# Autodesk Inventor assembly: Montagem
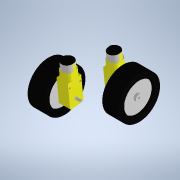
[picture p0: Inventor's stored thumbnail of the model, 180x180]
Saved by Autodesk Inventor 2020 (Build 240168000, 168)
## iProperties
Created: 2020-04-18
Part Number: Montagem
Document SubType Name: Assembly
Designer: eduardoADM
Author: eduardoADM
## Documents named in this file (3)
- C:\Users\eduardoADM\Desktop\robo\Montagem.iam
- C:\Users\eduardoADM\Desktop\robo\motorDC.ipt
- C:\Users\eduardoADM\Desktop\robo\roda.ipt
## Components (4 placed, 2 different names)
1. motorDC:1 — Coincidência:2
2. roda:1 — Coincidência:2
3. motorDC:2 — Coincidência:1
4. roda:2 — Coincidência:1
## Relationships (2: Mate 2)
- Coincidência:1 [Mate] (1.1 mm): motorDC:2 ↔ roda:2
- Coincidência:2 [Mate] (1.1 mm): motorDC:1 ↔ roda:1
